# Autodesk Inventor assembly: motorEaro
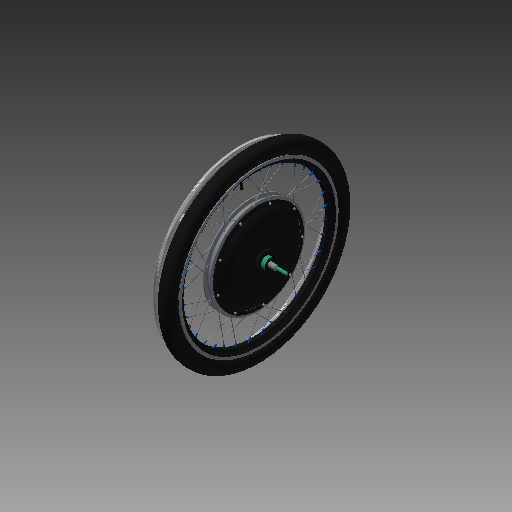
[picture p0: Inventor's stored thumbnail of the model, 512x512]
Saved by Autodesk Inventor 2017 (Build 210142000, 142)
## iProperties
Created: 2016-08-29
Part Number: motorEaro
Document SubType Name: Assembly
Designer: EriveltonDell
Author: EriveltonDell
## Documents named in this file (3)
- C:\Users\erive\Documents\GitHub\WheelchairDrawings\TEste\motorEaro.iam
- C:\Users\erive\Documents\GitHub\Power-Assisted-Wheelchair\Imported Components\Hub_Motor_MagicPie2_ASM\Hub_Motor_MagicPie2_ASM.iam
- C:\Users\erive\Documents\GitHub\WheelchairDrawings\TEste\Ciąg.iam
## Components (2 placed, 2 different names)
1. Hub_Motor_MagicPie2_ASM:1 [sub-assembly]
2. Ciąg:1 [sub-assembly]
## Relationships (1: Mate 1)
- [Mate]: Hub_Motor_MagicPie2_ASM:1 ↔ Ciąg:1
